# Autodesk Inventor assembly: Capping_Assembly
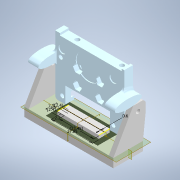
[picture p0: Inventor's stored thumbnail of the model, 180x180]
Saved by Autodesk Inventor 2022 (Build 260153000, 153)
## iProperties
Created: 2024-04-11
Part Number: Capping_Assembly
Document SubType Name: Assembly
Designer: Gotham City
Author: Gotham City
## Documents named in this file (6)
- E:\Xaar128\Capping_Assembly.iam
- C:\Users\Gotham City\Downloads\Holder - Printheadfixture(2).ipt
- E:\Xaar128\Part4.ipt
- E:\Xaar128\Capping_Insert.ipt
- E:\Xaar128\Part5.ipt
- E:\Xaar128\Part6.ipt
## Components (5 placed, 5 different names)
1. Holder - Printheadfixture(2):1 — Flush:1, Flush:2, Flush:3, Flush:4, Mate:2, Mate:3, Flush:6
2. Part4:1 — Flush:3
3. Capping_Insert:1 — Mate:1, Mate:2, Flush:9, Flush:10
4. Part5:1 — Mate:3, Flush:7, Flush:8, Flush:9
5. Part6:1 — Flush:10
## Relationships (12: Flush 9, Mate 3)
- Flush:1: Holder - Printheadfixture(2):1
- Flush:2: Holder - Printheadfixture(2):1
- Flush:3: Holder - Printheadfixture(2):1 ↔ Part4:1
- Flush:4 (2.27 mm): Holder - Printheadfixture(2):1
- Mate:1: Capping_Insert:1
- Mate:2 (2.85 mm): Holder - Printheadfixture(2):1 ↔ Capping_Insert:1
- Mate:3 (2.85 mm): Holder - Printheadfixture(2):1 ↔ Part5:1
- Flush:6 (-6.014 mm): Holder - Printheadfixture(2):1
- Flush:7 (-4.55 mm): Part5:1
- Flush:8: Part5:1
- Flush:9: Capping_Insert:1 ↔ Part5:1
- Flush:10: Capping_Insert:1 ↔ Part6:1
